# Autodesk Inventor assembly: 4t7000
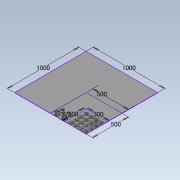
[picture p0: Inventor's stored thumbnail of the model, 180x180]
Saved by Autodesk Inventor 2020.3 (Build 243373000, 373)
## iProperties
Created: 2020-05-22
Part Number: 4t7000
Document SubType Name: Assembly
Designer: aoyama
Author: aoyama
## Documents named in this file (8)
- C:\Users\aoyam\Desktop\SRDC_local\Inventor\二年機\Geminiβ\4t7000.iam
- C:\Users\aoyam\Desktop\SRDC_local\Inventor\二年機\AL板サイズ測定板.ipt
- C:\Users\aoyam\Desktop\SRDC_local\Inventor\二年機\Geminiβ\脚\ネジクランク\クランク4t.ipt
- C:\Users\aoyam\Desktop\SRDC_local\Inventor\二年機\Geminiβ\脚\中間ユニット\脚中間フレームカム.ipt
- C:\Users\aoyam\Desktop\SRDC_local\Inventor\二年機\Geminiβ\腕\アームギアフレーム最内2.ipt
- C:\Users\aoyam\Desktop\SRDC_local\Inventor\二年機\Geminiβ\汎用部品\ｍ2歯数20ギアd5.98.ipt
- C:\Users\aoyam\Desktop\SRDC_local\Inventor\二年機\Geminiβ\汎用部品\m1歯数41ギアd5.98t4.ipt
- C:\Users\aoyam\Desktop\SRDC_local\Inventor\二年機\Geminiβ\エンドミルモデル.ipt
## Components (26 placed, 7 different names)
1. AL板サイズ測定板:1 — メイト:1, メイト:2, メイト:3, メイト:4, メイト:5, メイト:6, メイト:7, メイト:8, メイト:9
2. クランク4t:1 — メイト:7
3. クランク4t:2 — メイト:5
4. クランク4t:3 — メイト:3
5. クランク4t:4 — メイト:1
6. クランク4t:5 — メイト:2
7. クランク4t:6 — メイト:4
8. クランク4t:7 — メイト:6
9. クランク4t:8 — メイト:8
10. クランク4t:9
11. クランク4t:10
12. クランク4t:11
13. クランク4t:12
14. クランク4t:13
15. クランク4t:14
16. クランク4t:15
17. クランク4t:16
18. 脚中間フレームカム:1
19. 脚中間フレームカム:2
20. アームギアフレーム最内2:1
21. アームギアフレーム最内2:2
22. ｍ2歯数20ギアd5.98:1
23. ｍ2歯数20ギアd5.98:2
24. m1歯数41ギアd5.98t4:1
25. m1歯数41ギアd5.98t4:2
26. エンドミルモデル:1 — メイト:9
## Relationships (9: Mate 9)
- メイト:1 [Mate]: AL板サイズ測定板:1 ↔ クランク4t:4
- メイト:2 [Mate]: AL板サイズ測定板:1 ↔ クランク4t:5
- メイト:3 [Mate]: AL板サイズ測定板:1 ↔ クランク4t:3
- メイト:4 [Mate]: AL板サイズ測定板:1 ↔ クランク4t:6
- メイト:5 [Mate]: AL板サイズ測定板:1 ↔ クランク4t:2
- メイト:6 [Mate]: AL板サイズ測定板:1 ↔ クランク4t:7
- メイト:7 [Mate]: AL板サイズ測定板:1 ↔ クランク4t:1
- メイト:8 [Mate]: AL板サイズ測定板:1 ↔ クランク4t:8
- メイト:9 [Mate]: AL板サイズ測定板:1 ↔ エンドミルモデル:1
